# Autodesk Inventor assembly: frameWelded
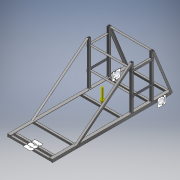
[picture p0: Inventor's stored thumbnail of the model, 180x180]
Saved by Autodesk Inventor 2018 (Build 220112000, 112)
## iProperties
Created: 2018-08-04
Part Number: frameWelded
Document SubType Name: Weldment
Designer: Cole Tucker
Weld Material: Welded Aluminum-6061
Mass: 17688.5 g
Surface Area: 10013 cm^2
Volume: 2260.26 cm^3
Density: 7.82589 g/cm^3
Author: Cole Tucker
## Documents named in this file (15)
- C:\Users\Cole Tucker\OneDrive\FRC-mxpProject\Cad\chassis\Inventor\frameWelded.iam
- C:\Users\Cole Tucker\OneDrive\FRC-mxpProject\Cad\chassis\Inventor\60in1.5Lch.ipt
- C:\Users\Cole Tucker\OneDrive\FRC-mxpProject\Cad\chassis\Inventor\22inSqTube.ipt
- C:\Users\Cole Tucker\OneDrive\FRC-mxpProject\Cad\chassis\Inventor\bearingplaterear.ipt
- C:\Users\Cole Tucker\OneDrive\FRC-mxpProject\Cad\chassis\Inventor\22in1.0Lch.ipt
- C:\Users\Cole Tucker\OneDrive\FRC-mxpProject\Cad\chassis\Inventor\36in1.0Lch.ipt
- C:\Users\Cole Tucker\OneDrive\FRC-mxpProject\Cad\chassis\Inventor\24.8in1.0Lch.ipt
- C:\Users\Cole Tucker\OneDrive\FRC-mxpProject\Cad\chassis\Inventor\11inbar.ipt
- C:\Users\Cole Tucker\OneDrive\FRC-mxpProject\Cad\chassis\Inventor\11in1.0lch.ipt
- C:\Users\Cole Tucker\OneDrive\FRC-mxpProject\Cad\chassis\Inventor\frameWelded\AIP\FEA\clef7olq8.fins
- C:\Users\Cole Tucker\OneDrive\FRC-mxpProject\Cad\chassis\Inventor\frameWelded\AIP\FEA\clef7olq8.fsat
- C:\Users\Cole Tucker\OneDrive\FRC-mxpProject\Cad\chassis\Inventor\frameWelded\AIP\FEA\clef7olq8.ftes
- C:\Users\Cole Tucker\OneDrive\FRC-mxpProject\Cad\chassis\Inventor\frameWelded\AIP\FEA\clef7olq8.fwiz
- C:\Users\Cole Tucker\OneDrive\FRC-mxpProject\Cad\chassis\Inventor\frameWelded\AIP\FEA\clef7olxc.fmsh
- C:\Users\Cole Tucker\OneDrive\FRC-mxpProject\Cad\chassis\Inventor\frameWelded\AIP\FEA\clef7olxd.fres
## Components (25 placed, 8 different names)
1. 60in1.5Lch:1 — Mate:1, Flush:9, Mate:4, Mate:5, Flush:15, Flush:17, Flush:18, Mate:11, Mate:12, Mate:27
2. 60in1.5Lch:2 — Flush:10, Mate:2, Mate:3, Mate:6, Flush:16, Flush:21, Flush:22, Mate:9, Mate:10, Mate:35
3. 22inSqTube:1 — Flush:1, Flush:2, Flush:3, Flush:4, Flush:5, Flush:6, Flush:7, Flush:8, Mate:1, Flush:9, Flush:10, Mate:2, Mate:3, Mate:4, Flush:11, Flush:12, Flush:13, Flush:14, Flush:19, Flush:20, Flush:23, Flush:24, Flush:28, Flush:29
4. 22inSqTube:2 — Flush:1, Flush:5, Flush:11
5. 22inSqTube:3 — Flush:2, Flush:6, Flush:12, Mate:20, Mate:24
6. 22inSqTube:4 — Flush:3, Flush:7, Flush:14
7. 22inSqTube:5 — Flush:4, Flush:8, Flush:13, Mate:7, Mate:8, Mate:33
8. bearingplaterear:1 — Mate:5, Flush:15, Mate:8
9. bearingplaterear:2 — Mate:6, Flush:16, Mate:7
10. 22inSqTube:6 — Flush:22, Flush:23, Mate:9, Mate:17, Mate:18, Mate:23, Mate:25, Mate:26, Mate:39, Flush:36, Flush:37, Flush:38, Mate:40, Flush:39
11. 22inSqTube:7 — Flush:21, Flush:24, Mate:10, Mate:32
12. 22inSqTube:8 — Flush:18, Flush:20, Mate:12, Mate:13, Flush:25, Mate:14, Mate:30
13. 22inSqTube:9 — Flush:17, Flush:19, Mate:11, Mate:15, Flush:26, Mate:16, Mate:19, Mate:21, Mate:22, Mate:37, Flush:32, Flush:33, Mate:41, Flush:40, Flush:41
14. 22in1.0Lch:1 — Mate:15, Flush:26, Mate:16, Flush:27
15. 22in1.0Lch:2 — Mate:13, Flush:25, Mate:14, Mate:28, Mate:29, Mate:31, Mate:34
16. 22in1.0Lch:3 — Mate:17, Flush:27, Mate:18
17. 36in1.0Lch:1 — Mate:19, Mate:20, Mate:21, Mate:22
18. 36in1.0Lch:2 — Mate:23, Mate:24, Mate:25, Mate:26
19. 24.8in1.0Lch:1 — Mate:27, Mate:28, Mate:29, Mate:30
20. 24.8in1.0Lch:2 — Mate:31, Mate:32, Mate:33, Mate:34
21. 22inSqTube:10 — Mate:35, Flush:28, Flush:29
22. 11inbar:2 — Mate:37, Flush:32, Flush:33
23. 11inbar:3 — Mate:39, Flush:36, Flush:37
24. 11in1.0lch:1 — Mate:41, Flush:40, Flush:41
25. 11in1.0lch:2 — Flush:38, Mate:40, Flush:39
## Relationships (76: Mate 39, Flush 37)
- Flush:1: 22inSqTube:1 ↔ 22inSqTube:2
- Flush:2: 22inSqTube:1 ↔ 22inSqTube:3
- Flush:3: 22inSqTube:1 ↔ 22inSqTube:4
- Flush:4: 22inSqTube:1 ↔ 22inSqTube:5
- Flush:5: 22inSqTube:1 ↔ 22inSqTube:2
- Flush:6: 22inSqTube:1 ↔ 22inSqTube:3
- Flush:7: 22inSqTube:1 ↔ 22inSqTube:4
- Flush:8: 22inSqTube:1 ↔ 22inSqTube:5
- Mate:1: 60in1.5Lch:1 ↔ 22inSqTube:1
- Flush:9: 60in1.5Lch:1 ↔ 22inSqTube:1
- Flush:10: 60in1.5Lch:2 ↔ 22inSqTube:1
- Mate:2: 60in1.5Lch:2 ↔ 22inSqTube:1
- Mate:3: 60in1.5Lch:2 ↔ 22inSqTube:1
- Mate:4: 60in1.5Lch:1 ↔ 22inSqTube:1
- Flush:11 (50.8 mm): 22inSqTube:1 ↔ 22inSqTube:2
- Flush:12 (304.8 mm): 22inSqTube:1 ↔ 22inSqTube:3
- Flush:13 (1498.6 mm): 22inSqTube:1 ↔ 22inSqTube:5
- Flush:14 (914.4 mm): 22inSqTube:1 ↔ 22inSqTube:4
- Mate:5: 60in1.5Lch:1 ↔ bearingplaterear:1
- Flush:15: 60in1.5Lch:1 ↔ bearingplaterear:1
- Mate:6: 60in1.5Lch:2 ↔ bearingplaterear:2
- Flush:16: 60in1.5Lch:2 ↔ bearingplaterear:2
- Mate:7 (-127 mm): 22inSqTube:5 ↔ bearingplaterear:2
- Mate:8 (-127 mm): 22inSqTube:5 ↔ bearingplaterear:1
- Flush:17: 60in1.5Lch:1 ↔ 22inSqTube:9
- Flush:18: 60in1.5Lch:1 ↔ 22inSqTube:8
- Flush:19 (1016 mm): 22inSqTube:1 ↔ 22inSqTube:9
- Flush:20 (1270 mm): 22inSqTube:1 ↔ 22inSqTube:8
- Flush:21: 60in1.5Lch:2 ↔ 22inSqTube:7
- Flush:22: 60in1.5Lch:2 ↔ 22inSqTube:6
- Flush:23 (1016 mm): 22inSqTube:1 ↔ 22inSqTube:6
- Flush:24 (1270 mm): 22inSqTube:1 ↔ 22inSqTube:7
- Mate:9: 60in1.5Lch:2 ↔ 22inSqTube:6
- Mate:10: 60in1.5Lch:2 ↔ 22inSqTube:7
- Mate:11: 60in1.5Lch:1 ↔ 22inSqTube:9
- Mate:12: 60in1.5Lch:1 ↔ 22inSqTube:8
- Mate:13: 22inSqTube:8 ↔ 22in1.0Lch:2
- Flush:25: 22inSqTube:8 ↔ 22in1.0Lch:2
- Mate:14: 22inSqTube:8 ↔ 22in1.0Lch:2
- Mate:15: 22inSqTube:9 ↔ 22in1.0Lch:1
- Flush:26 (76.2 mm): 22inSqTube:9 ↔ 22in1.0Lch:1
- Mate:16: 22inSqTube:9 ↔ 22in1.0Lch:1
- Mate:17: 22inSqTube:6 ↔ 22in1.0Lch:3
- Flush:27 (279.4 mm): 22in1.0Lch:1 ↔ 22in1.0Lch:3
- Mate:18: 22inSqTube:6 ↔ 22in1.0Lch:3
- Mate:19: 22inSqTube:9 ↔ 36in1.0Lch:1
- Mate:20: 22inSqTube:3 ↔ 36in1.0Lch:1
- Mate:21: 22inSqTube:9 ↔ 36in1.0Lch:1
- Mate:22: 22inSqTube:9 ↔ 36in1.0Lch:1
- Mate:23: 22inSqTube:6 ↔ 36in1.0Lch:2
- Mate:24: 22inSqTube:3 ↔ 36in1.0Lch:2
- Mate:25: 22inSqTube:6 ↔ 36in1.0Lch:2
- Mate:26: 22inSqTube:6 ↔ 36in1.0Lch:2
- Mate:27: 60in1.5Lch:1 ↔ 24.8in1.0Lch:1
- Mate:28: 22in1.0Lch:2 ↔ 24.8in1.0Lch:1
- Mate:29: 22in1.0Lch:2 ↔ 24.8in1.0Lch:1
- Mate:30: 22inSqTube:8 ↔ 24.8in1.0Lch:1
- Mate:31: 22in1.0Lch:2 ↔ 24.8in1.0Lch:2
- Mate:32: 22inSqTube:7 ↔ 24.8in1.0Lch:2
- Mate:33: 22inSqTube:5 ↔ 24.8in1.0Lch:2
- Mate:34: 22in1.0Lch:2 ↔ 24.8in1.0Lch:2
- Mate:35: 60in1.5Lch:2 ↔ 22inSqTube:10
- Flush:28: 22inSqTube:1 ↔ 22inSqTube:10
- Flush:29 (1270 mm): 22inSqTube:1 ↔ 22inSqTube:10
- Mate:37: 22inSqTube:9 ↔ 11inbar:2
- Flush:32: 22inSqTube:9 ↔ 11inbar:2
- Flush:33 (355.6 mm): 22inSqTube:9 ↔ 11inbar:2
- Mate:39: 22inSqTube:6 ↔ 11inbar:3
- Flush:36: 22inSqTube:6 ↔ 11inbar:3
- Flush:37 (355.6 mm): 22inSqTube:6 ↔ 11inbar:3
- Flush:38: 22inSqTube:6 ↔ 11in1.0lch:2
- Mate:40: 22inSqTube:6 ↔ 11in1.0lch:2
- Flush:39 (76.2 mm): 22inSqTube:6 ↔ 11in1.0lch:2
- Mate:41: 22inSqTube:9 ↔ 11in1.0lch:1
- Flush:40: 22inSqTube:9 ↔ 11in1.0lch:1
- Flush:41 (76.2 mm): 22inSqTube:9 ↔ 11in1.0lch:1
## Named parameters: sa_0 = 2.50435e-10, sa_1 = -44482.2, sa_2 = -1.30867e-09
note: some values were not read from the file. Shown as the stored number, unit unknown: "sa_0", "sa_1", "sa_2".
